# Autodesk Inventor assembly: Oval Wardrobe Bar
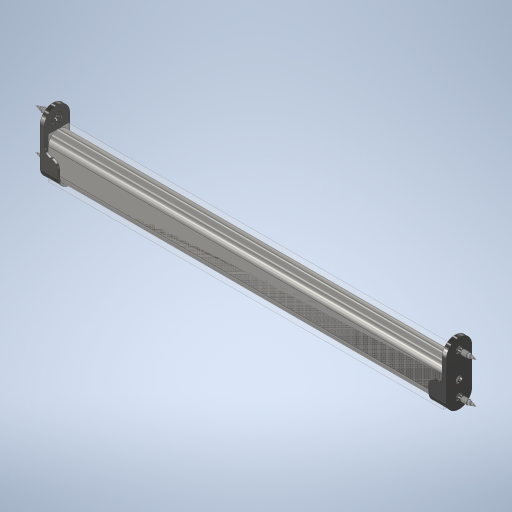
[picture p0: Inventor's stored thumbnail of the model, 512x512]
Saved by Autodesk Inventor 2024 (Build 280153000, 153)
## iProperties
Created: 2015-03-09
Part Number: Oval Wardrobe Bar
Document SubType Name: Assembly
Designer: SauliusD
Description: Oval Wardrobe Bar with Fixtures
Author: SauliusD
## Documents named in this file (4)
- C:\W4INV 2024 Design\iBOX LIBRARY\Wardrobe Accesories\Oval Wardrobe Bar\Oval Wardrobe Bar.iam
- C:\W4INV 2024 Design\iBOX LIBRARY\Wardrobe Accesories\Oval Wardrobe Bar\Oval Wardrobe Bar.ipt
- C:\W4INV 2024 Design\iBOX LIBRARY\Wardrobe Accesories\Oval Wardrobe Bar\Fixture for the Oval Bar.ipt
- C:\W4INV 2024 Design\iBOX LIBRARY\Wardrobe Accesories\Oval Wardrobe Bar\Oval Wardrobe Bar Skeleton.ipt
## Components (4 placed, 4 different names)
1. @Skeleton — Flush:2, Flush:3, Flush:4
2. Oval Wardrobe Bar:1 — Mate:1, Mate:2, Tangent:1, Tangent:2
3. @Fixture for the Oval Bar Left — Mate:1, Flush:1, Tangent:1
4. @Fixture for the Oval Bar Right — Mate:2, Mate:3, Tangent:2
## Relationships (9: Flush 4, Mate 3, Tangent 2)
- Mate:1 (1 mm): Oval Wardrobe Bar:1 ↔ @Fixture for the Oval Bar Left
- Mate:2 (1 mm): Oval Wardrobe Bar:1 ↔ @Fixture for the Oval Bar Right
- Flush:1: @Fixture for the Oval Bar Left
- Mate:3: @Fixture for the Oval Bar Right
- Tangent:1: Oval Wardrobe Bar:1 ↔ @Fixture for the Oval Bar Left
- Tangent:2: Oval Wardrobe Bar:1 ↔ @Fixture for the Oval Bar Right
- Flush:2: @Skeleton
- Flush:3: @Skeleton
- Flush:4: @Skeleton
